# Autodesk Inventor assembly: assem_palm_test_v1
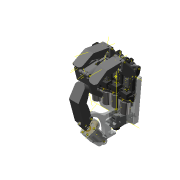
[picture p0: Inventor's stored thumbnail of the model, 180x180]
Saved by Autodesk Inventor 2014 (Build 180170000, 170)
## iProperties
Created: 2015-05-07
Part Number: assem_palm_test_v1
Document SubType Name: Assembly
Designer: Martin
Author: Martin
## Documents named in this file (16)
- C:\Users\Martin\Dropbox\biohand-mec\biohand_v1\palm\assem_palm_test_v3.iam
- C:\Users\Martin\Dropbox\biohand-mec\biohand_v1\fingers\index\assem_finger_index.iam
- C:\Users\Martin\Dropbox\biohand-mec\biohand_v1\fingers\middle\assem_finger_middle.iam
- C:\Users\Martin\Dropbox\biohand-mec\biohand_v1\fingers\ring\assem_finger_ring.iam
- C:\Users\Martin\Dropbox\biohand-mec\biohand_v1\fingers\pinky\assem_finger_pinky.iam
- C:\Users\Martin\Dropbox\biohand-mec\biohand_v1\palm\palm_back_v5.ipt
- C:\Users\Martin\Dropbox\biohand-mec\biohand_v1\misc\micro_servo.ipt
- C:\Users\Martin\Dropbox\biohand-mec\biohand_v1\palm\servo_clamp_v2.ipt
- C:\Users\Martin\Dropbox\biohand-mec\biohand_v1\misc\bearing_10_4_3.ipt
- C:\Users\Martin\Dropbox\biohand-mec\biohand_v1\fingers\thumb\thumb_base_v2.ipt
- C:\Users\Martin\Dropbox\biohand-mec\biohand_v1\misc\m3_10_screw.ipt
- C:\Users\Martin\Dropbox\biohand-mec\biohand_v1\fingers\thumb\assem_finger_thumb_linact_v3.iam
- C:\Users\Martin\Dropbox\biohand-mec\biohand_v1\fingers\thumb\assem_linact_thumb_rod.iam
- C:\Users\Martin\Dropbox\biohand-mec\biohand_v1\fingers\thumb\thumb_phalanx_v2_a.ipt
- C:\Users\Martin\Dropbox\biohand-mec\biohand_v1\misc\servo_square_pot.ipt
- C:\Users\Martin\Dropbox\biohand-mec\biohand_v1\misc\m2_8_screw.ipt
## Components (19 placed, 15 different names)
1. palm_back_v5:1 — Flush:1, Flush:2, Flush:3, Mate:1, Mate:2, Mate:3, Mate:4, Mate:5, Mate:6, Mate:7, Mate:8, Mate:9, Mate:10, Mate:11, Mate:12, Mate:13, Angle:1, Mate:17, Mate:18, Mate:19, Mate:20
2. assem_finger_index:1 [sub-assembly] — Mate:1, Mate:2, Mate:3
3. assem_finger_middle:1 [sub-assembly] — Mate:4, Mate:7, Mate:10
4. assem_finger_ring:1 [sub-assembly] — Mate:5, Mate:8, Mate:11
5. assem_finger_pinky:1 [sub-assembly] — Mate:6, Mate:9, Mate:12
6. micro_servo:1 — Mate:13, Angle:1, Mate:22
7. bearing_10_4_3:1 — Insert:12
8. thumb_base_v2:2 — Angle:2, Insert:4, Insert:5, Mate:18, Insert:13, Insert:14
9. m3_10_screw:1 — Insert:13
10. assem_finger_thumb_linact_v3:1 [sub-assembly] — Insert:4, Mate:15, Angle:3, Insert:10, Insert:11
11. assem_linact_thumb_rod:1 [sub-assembly] — Mate:15, Angle:3, Mate:16
12. servo_square_pot:1 — Insert:7, Angle:4
13. m2_8_screw:1 — Insert:6
14. m2_8_screw:2 — Insert:9
15. m2_8_screw:3 — Insert:8
16. thumb_phalanx_v2_a:1 — Insert:5, Mate:16, Insert:6, Insert:7, Angle:4, Insert:8, Insert:9
17. m2_8_screw:4 — Insert:10
18. m2_8_screw:5 — Insert:11
19. servo_clamp_v2:1 — Mate:19, Angle:5, Mate:20, Insert:12, Mate:22, Insert:14
## Relationships (39: Mate 20, Insert 11, Angle 5, Flush 3)
- Flush:1: palm_back_v5:1
- Flush:2: palm_back_v5:1
- Flush:3: palm_back_v5:1
- Mate:1: palm_back_v5:1 ↔ assem_finger_index:1
- Mate:2: palm_back_v5:1 ↔ assem_finger_index:1
- Mate:3: palm_back_v5:1 ↔ assem_finger_index:1
- Mate:4: palm_back_v5:1 ↔ assem_finger_middle:1
- Mate:5: palm_back_v5:1 ↔ assem_finger_ring:1
- Mate:6: palm_back_v5:1 ↔ assem_finger_pinky:1
- Mate:7: palm_back_v5:1 ↔ assem_finger_middle:1
- Mate:8: palm_back_v5:1 ↔ assem_finger_ring:1
- Mate:9: palm_back_v5:1 ↔ assem_finger_pinky:1
- Mate:10: palm_back_v5:1 ↔ assem_finger_middle:1
- Mate:11: palm_back_v5:1 ↔ assem_finger_ring:1
- Mate:12: palm_back_v5:1 ↔ assem_finger_pinky:1
- Mate:13: palm_back_v5:1 ↔ micro_servo:1
- Angle:1 (0 deg): palm_back_v5:1 ↔ micro_servo:1
- Angle:2 (0 deg): thumb_base_v2:2
- Insert:4 (0.5 mm): thumb_base_v2:2 ↔ assem_finger_thumb_linact_v3:1
- Mate:15: assem_finger_thumb_linact_v3:1 ↔ assem_linact_thumb_rod:1
- Angle:3 (0 deg): assem_finger_thumb_linact_v3:1 ↔ assem_linact_thumb_rod:1
- Insert:5 (0.5 mm): thumb_base_v2:2 ↔ thumb_phalanx_v2_a:1
- Mate:16: assem_linact_thumb_rod:1 ↔ thumb_phalanx_v2_a:1
- Insert:6: m2_8_screw:1 ↔ thumb_phalanx_v2_a:1
- Insert:7: servo_square_pot:1 ↔ thumb_phalanx_v2_a:1
- Angle:4 (180 deg): servo_square_pot:1 ↔ thumb_phalanx_v2_a:1
- Insert:8: m2_8_screw:3 ↔ thumb_phalanx_v2_a:1
- Insert:9: m2_8_screw:2 ↔ thumb_phalanx_v2_a:1
- Insert:10: assem_finger_thumb_linact_v3:1 ↔ m2_8_screw:4
- Insert:11: assem_finger_thumb_linact_v3:1 ↔ m2_8_screw:5
- Mate:17: palm_back_v5:1
- Mate:18: palm_back_v5:1 ↔ thumb_base_v2:2
- Mate:19: palm_back_v5:1 ↔ servo_clamp_v2:1
- Angle:5 (0 deg): servo_clamp_v2:1
- Mate:20: palm_back_v5:1 ↔ servo_clamp_v2:1
- Insert:12: bearing_10_4_3:1 ↔ servo_clamp_v2:1
- Insert:13: thumb_base_v2:2 ↔ m3_10_screw:1
- Mate:22: micro_servo:1 ↔ servo_clamp_v2:1
- Insert:14 (0.25 mm): thumb_base_v2:2 ↔ servo_clamp_v2:1
